# Autodesk Inventor assembly: Shuttle
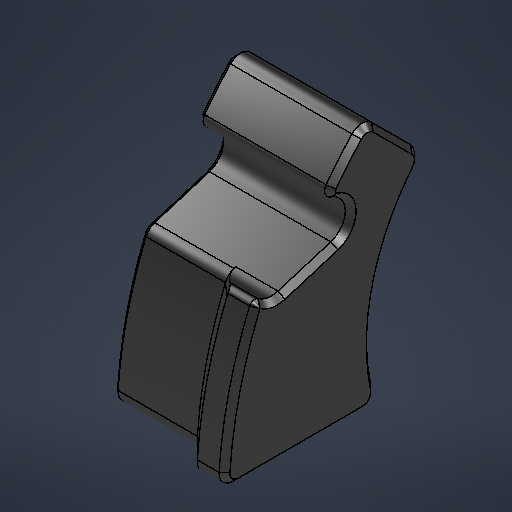
[picture p0: Inventor's stored thumbnail of the model, 512x512]
Saved by Autodesk Inventor 2026 (Build 300175050, 175E)
## iProperties
Created: 2025-05-11
Part Number: Shuttle
Document SubType Name: Assembly
Designer: Joshua Eah
Author: Joshua Eah
## Documents named in this file (3)
- C:\Users\Joshua Eah\Documents\GitHub\Voron-0\CAD\Master Assembly\Toolhead\Subassemblies\Shuttle.iam
- C:\Users\Joshua Eah\Documents\GitHub\Voron-0\CAD\Master Assembly\Hardware\M3 Threaded Insert.ipt
- C:\Users\Joshua Eah\Documents\GitHub\Voron-0\CAD\Master Assembly\Toolhead\Parts\Shuttle.ipt
## Components (2 placed, 2 different names)
1. M3 Threaded Insert:1 — Insert:1
2. Shuttle:1 — Insert:1
## Relationships (1: Insert 1)
- Insert:1: M3 Threaded Insert:1 ↔ Shuttle:1
